# Autodesk Inventor assembly: Objective
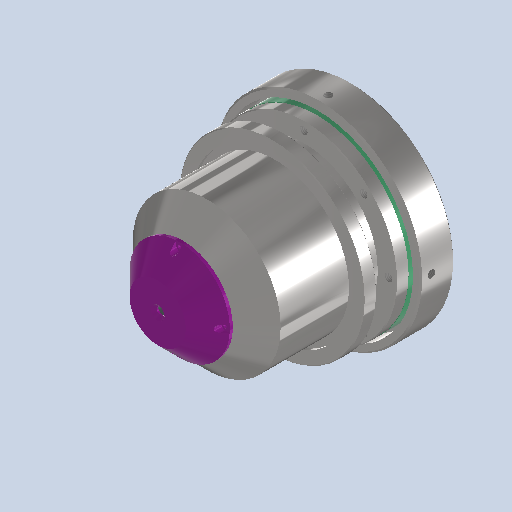
[picture p0: Inventor's stored thumbnail of the model, 512x512]
Saved by Autodesk Inventor 2023 (Build 270158000, 158)
## iProperties
Created: 2022-03-30
Part Number: Objective
Document SubType Name: Assembly
Designer: Vinicius Miguel
Author: Vinicius Miguel
## Documents named in this file (8)
- P:\SEM-Mechanical\Objective.iam
- P:\SEM-Mechanical\001.ipt
- P:\SEM-Mechanical\002.ipt
- P:\SEM-Mechanical\003.ipt
- P:\SEM-Mechanical\004.ipt
- P:\SEM-Mechanical\005.ipt
- P:\SEM-Mechanical\006.ipt
- P:\SEM-Mechanical\007.ipt
## Components (7 placed, 7 different names)
1. 001:1 — Mate:1, Flush:1, Flush:2, Mate:3
2. 002:1 — Mate:4
3. 003:1 — Mate:2, Mate:3, Flush:3, Mate:8
4. 004:1 — Mate:5, Mate:6
5. 005:1 — Mate:4, Mate:5, Mate:6, Mate:7, Mate:8, Mate:10
6. 006:1 — Mate:9, Mate:10, Mate:11, Flush:4
7. 007:1 — Mate:11
## Relationships (15: Mate 11, Flush 4)
- Mate:1: 001:1
- Flush:1: 001:1
- Flush:2: 001:1
- Mate:2: 003:1
- Mate:3: 001:1 ↔ 003:1
- Flush:3: 003:1
- Mate:4: 002:1 ↔ 005:1
- Mate:5: 004:1 ↔ 005:1
- Mate:6: 004:1 ↔ 005:1
- Mate:7: 005:1
- Mate:8: 003:1 ↔ 005:1
- Mate:9: 006:1
- Mate:10: 005:1 ↔ 006:1
- Mate:11: 006:1 ↔ 007:1
- Flush:4: 006:1
